# Autodesk Inventor assembly: Cage
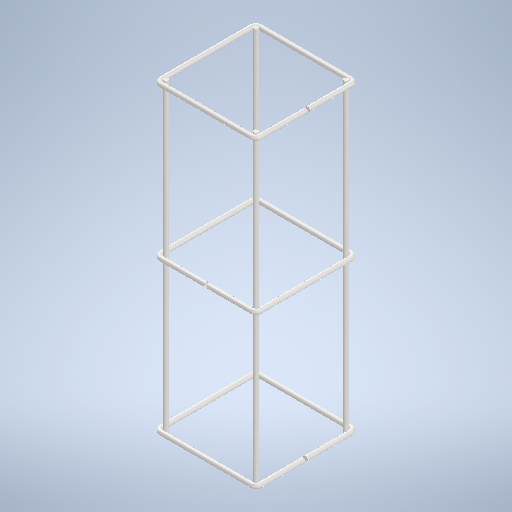
[picture p0: Inventor's stored thumbnail of the model, 512x512]
Saved by Autodesk Inventor 2025 (Build 290162010, 162A)
## iProperties
Created: 2024-09-07
Part Number: Cage
Document SubType Name: Assembly
Designer: Tom
Author: Tom
## Documents named in this file (3)
- C:\Users\Tom\Documents\Inventor\Mobility\Additional_Building\Cage.iam
- C:\Users\Tom\Documents\Inventor\Mobility\Additional_Building\Ring_Of_Rebar.ipt
- C:\Users\Tom\Documents\Inventor\Mobility\Additional_Building\Rebar_With_Length_Of_34_Inches.ipt
## Components (7 placed, 2 different names)
1. Ring_Of_Rebar:1 — Tangent:1, Tangent:2, Tangent:3, Mate:1, Mate:2, Mate:3, Tangent:7, Tangent:8, Tangent:9, Mate:4, Tangent:10, Tangent:11, Tangent:12, Tangent:13, Tangent:14, Tangent:15, Flush:1, Flush:2
2. Rebar_With_Length_Of_34_Inches:1 — Mate:3, Tangent:7, Tangent:8, Tangent:9, Tangent:22, Tangent:23, Tangent:24, Tangent:37, Tangent:38, Tangent:39
3. Rebar_With_Length_Of_34_Inches:2 — Tangent:1, Tangent:2, Tangent:3, Mate:1, Tangent:17, Tangent:20, Tangent:21, Tangent:34, Tangent:35, Tangent:36
4. Rebar_With_Length_Of_34_Inches:3 — Mate:4, Tangent:10, Tangent:11, Tangent:12, Mate:5, Tangent:16, Tangent:18, Tangent:19, Mate:6, Tangent:28, Tangent:29, Tangent:30
5. Rebar_With_Length_Of_34_Inches:4 — Mate:2, Tangent:13, Tangent:14, Tangent:15, Tangent:25, Tangent:26, Tangent:27, Tangent:31, Tangent:32, Tangent:33
6. Ring_Of_Rebar:2 — Mate:5, Tangent:16, Tangent:17, Tangent:18, Tangent:19, Tangent:20, Tangent:21, Tangent:22, Tangent:23, Tangent:24, Tangent:25, Tangent:26, Tangent:27
7. Ring_Of_Rebar:3 — Tangent:28, Tangent:29, Tangent:30, Tangent:31, Tangent:32, Tangent:33, Tangent:34, Tangent:35, Tangent:36, Tangent:37, Tangent:38, Tangent:39, Mate:7
## Relationships (45: Tangent 36, Mate 7, Flush 2)
- Tangent:1: Ring_Of_Rebar:1 ↔ Rebar_With_Length_Of_34_Inches:2
- Tangent:2: Ring_Of_Rebar:1 ↔ Rebar_With_Length_Of_34_Inches:2
- Tangent:3: Ring_Of_Rebar:1 ↔ Rebar_With_Length_Of_34_Inches:2
- Mate:1 (-6.35 mm): Ring_Of_Rebar:1 ↔ Rebar_With_Length_Of_34_Inches:2
- Mate:2 (-6.35 mm): Ring_Of_Rebar:1 ↔ Rebar_With_Length_Of_34_Inches:4
- Mate:3 (-6.35 mm): Ring_Of_Rebar:1 ↔ Rebar_With_Length_Of_34_Inches:1
- Tangent:7: Ring_Of_Rebar:1 ↔ Rebar_With_Length_Of_34_Inches:1
- Tangent:8: Ring_Of_Rebar:1 ↔ Rebar_With_Length_Of_34_Inches:1
- Tangent:9: Ring_Of_Rebar:1 ↔ Rebar_With_Length_Of_34_Inches:1
- Mate:4 (-6.35 mm): Ring_Of_Rebar:1 ↔ Rebar_With_Length_Of_34_Inches:3
- Tangent:10: Ring_Of_Rebar:1 ↔ Rebar_With_Length_Of_34_Inches:3
- Tangent:11: Ring_Of_Rebar:1 ↔ Rebar_With_Length_Of_34_Inches:3
- Tangent:12: Ring_Of_Rebar:1 ↔ Rebar_With_Length_Of_34_Inches:3
- Tangent:13: Ring_Of_Rebar:1 ↔ Rebar_With_Length_Of_34_Inches:4
- Tangent:14: Ring_Of_Rebar:1 ↔ Rebar_With_Length_Of_34_Inches:4
- Tangent:15: Ring_Of_Rebar:1 ↔ Rebar_With_Length_Of_34_Inches:4
- Mate:5 (-6.35 mm): Rebar_With_Length_Of_34_Inches:3 ↔ Ring_Of_Rebar:2
- Tangent:16: Rebar_With_Length_Of_34_Inches:3 ↔ Ring_Of_Rebar:2
- Tangent:17: Rebar_With_Length_Of_34_Inches:2 ↔ Ring_Of_Rebar:2
- Tangent:18: Rebar_With_Length_Of_34_Inches:3 ↔ Ring_Of_Rebar:2
- Tangent:19: Rebar_With_Length_Of_34_Inches:3 ↔ Ring_Of_Rebar:2
- Tangent:20: Rebar_With_Length_Of_34_Inches:2 ↔ Ring_Of_Rebar:2
- Tangent:21: Rebar_With_Length_Of_34_Inches:2 ↔ Ring_Of_Rebar:2
- Tangent:22: Rebar_With_Length_Of_34_Inches:1 ↔ Ring_Of_Rebar:2
- Tangent:23: Rebar_With_Length_Of_34_Inches:1 ↔ Ring_Of_Rebar:2
- Tangent:24: Rebar_With_Length_Of_34_Inches:1 ↔ Ring_Of_Rebar:2
- Tangent:25: Rebar_With_Length_Of_34_Inches:4 ↔ Ring_Of_Rebar:2
- Tangent:26: Rebar_With_Length_Of_34_Inches:4 ↔ Ring_Of_Rebar:2
- Tangent:27: Rebar_With_Length_Of_34_Inches:4 ↔ Ring_Of_Rebar:2
- Mate:6: Rebar_With_Length_Of_34_Inches:3
- Flush:1: Ring_Of_Rebar:1
- Flush:2: Ring_Of_Rebar:1
- Tangent:28: Rebar_With_Length_Of_34_Inches:3 ↔ Ring_Of_Rebar:3
- Tangent:29: Rebar_With_Length_Of_34_Inches:3 ↔ Ring_Of_Rebar:3
- Tangent:30: Rebar_With_Length_Of_34_Inches:3 ↔ Ring_Of_Rebar:3
- Tangent:31: Rebar_With_Length_Of_34_Inches:4 ↔ Ring_Of_Rebar:3
- Tangent:32: Rebar_With_Length_Of_34_Inches:4 ↔ Ring_Of_Rebar:3
- Tangent:33: Rebar_With_Length_Of_34_Inches:4 ↔ Ring_Of_Rebar:3
- Tangent:34: Rebar_With_Length_Of_34_Inches:2 ↔ Ring_Of_Rebar:3
- Tangent:35: Rebar_With_Length_Of_34_Inches:2 ↔ Ring_Of_Rebar:3
- Tangent:36: Rebar_With_Length_Of_34_Inches:2 ↔ Ring_Of_Rebar:3
- Tangent:37: Rebar_With_Length_Of_34_Inches:1 ↔ Ring_Of_Rebar:3
- Tangent:38: Rebar_With_Length_Of_34_Inches:1 ↔ Ring_Of_Rebar:3
- Tangent:39: Rebar_With_Length_Of_34_Inches:1 ↔ Ring_Of_Rebar:3
- Mate:7 (431.8 mm): Ring_Of_Rebar:3
